# Autodesk Inventor assembly: tendeur_block
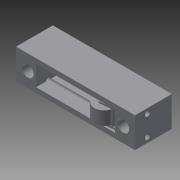
[picture p0: Inventor's stored thumbnail of the model, 180x180]
Saved by Autodesk Inventor 2014 SP1 (Build 180222100, 222)
## iProperties
Created: 2015-09-12
Part Number: tendeur_block
Document SubType Name: Assembly
Designer: astralien3000
Author: astralien3000
## Documents named in this file (4)
- C:\Users\astralien3000\Desktop\ceres\meca\v2016\tendeur_block.iam
- C:\Users\astralien3000\Desktop\ceres\meca\v2016\tendeur_complet.iam
- C:\Users\astralien3000\Desktop\ceres\meca\v2016\tendeur_base_low.ipt
- C:\Users\astralien3000\Desktop\ceres\meca\v2016\tendeur_base_up.ipt
## Components (3 placed, 3 different names)
1. tendeur_complet:1 [sub-assembly] — Placage:4, Placage:5
2. tendeur_base_low:1 — Placage:1, Placage:2, Placage:3, Placage:5
3. tendeur_base_up:1 — Placage:1, Placage:2, Placage:3, Placage:4
## Relationships (5: Mate 5)
- Placage:1 [Mate]: tendeur_base_low:1 ↔ tendeur_base_up:1
- Placage:2 [Mate]: tendeur_base_low:1 ↔ tendeur_base_up:1
- Placage:3 [Mate]: tendeur_base_low:1 ↔ tendeur_base_up:1
- Placage:4 [Mate]: tendeur_complet:1 ↔ tendeur_base_up:1
- Placage:5 [Mate] (0.5 mm): tendeur_complet:1 ↔ tendeur_base_low:1
